# Autodesk Inventor assembly: Gantry Assm
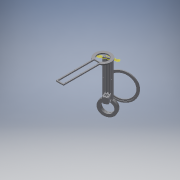
[picture p0: Inventor's stored thumbnail of the model, 180x180]
Saved by Autodesk Inventor 2016 (Build 200138000, 138)
## iProperties
Created: 2016-04-22
Part Number: Gantry Assm
Document SubType Name: Assembly
Designer: rubenjm
Author: rubenjm
## Documents named in this file (8)
- C:\Users\rubenjm\Documents\To Transfer\2k16 Spring\RME\GGC\V2\Gantry Assm.iam
- C:\Users\rubenjm\Documents\To Transfer\2k16 Spring\RME\GGC\V2\NEMA23 Motor.ipt
- C:\Users\rubenjm\Documents\To Transfer\2k16 Spring\RME\GGC\V2\Arm Top Layer.ipt
- C:\Users\rubenjm\Documents\To Transfer\2k16 Spring\RME\GGC\V2\Motor Bracket.ipt
- C:\Users\rubenjm\Documents\To Transfer\2k16 Spring\RME\GGC\V2\Unthreaded Rod.ipt
- C:\Users\rubenjm\Documents\To Transfer\2k16 Spring\RME\GGC\V2\Turntable.ipt
- C:\Users\rubenjm\Documents\To Transfer\2k16 Spring\RME\GGC\V2\Arm Layer 2.ipt
- C:\Users\rubenjm\Documents\To Transfer\2k16 Spring\RME\GGC\V2\Arm Layer 3.ipt
## Components (9 placed, 7 different names)
1. Arm Top Layer:1 — Mate:7, Mate:8, Mate:9, Mate:12, Mate:16, Mate:17, Mate:18, Mate:21, Mate:22
2. NEMA23 Motor:1 — Mate:4, Mate:5, Mate:6
3. Motor Bracket:1 — Mate:4, Mate:5, Mate:6, Mate:7, Mate:8, Mate:9, Mate:10, Mate:11
4. Unthreaded Rod:1 — Mate:10, Mate:19
5. Unthreaded Rod:2 — Mate:11, Mate:20
6. Turntable:1 — Mate:12
7. Arm Layer 2:1 — Mate:16, Mate:17, Mate:18, Mate:19, Mate:20, Mate:21, Mate:22, Mate:23, Mate:24, Mate:25
8. Arm Layer 2:2 — Mate:23, Mate:24, Mate:25
9. Arm Layer 3:1
## Relationships (19: Mate 19)
- Mate:4: NEMA23 Motor:1 ↔ Motor Bracket:1
- Mate:5: NEMA23 Motor:1 ↔ Motor Bracket:1
- Mate:6: NEMA23 Motor:1 ↔ Motor Bracket:1
- Mate:7: Arm Top Layer:1 ↔ Motor Bracket:1
- Mate:8: Arm Top Layer:1 ↔ Motor Bracket:1
- Mate:9: Arm Top Layer:1 ↔ Motor Bracket:1
- Mate:10: Motor Bracket:1 ↔ Unthreaded Rod:1
- Mate:11: Motor Bracket:1 ↔ Unthreaded Rod:2
- Mate:12: Arm Top Layer:1 ↔ Turntable:1
- Mate:16: Arm Top Layer:1 ↔ Arm Layer 2:1
- Mate:17: Arm Top Layer:1 ↔ Arm Layer 2:1
- Mate:18: Arm Top Layer:1 ↔ Arm Layer 2:1
- Mate:19: Unthreaded Rod:1 ↔ Arm Layer 2:1
- Mate:20: Unthreaded Rod:2 ↔ Arm Layer 2:1
- Mate:21: Arm Top Layer:1 ↔ Arm Layer 2:1
- Mate:22: Arm Top Layer:1 ↔ Arm Layer 2:1
- Mate:23: Arm Layer 2:1 ↔ Arm Layer 2:2
- Mate:24: Arm Layer 2:1 ↔ Arm Layer 2:2
- Mate:25: Arm Layer 2:1 ↔ Arm Layer 2:2
